# Autodesk Inventor assembly: Ariadna_&_Konarm
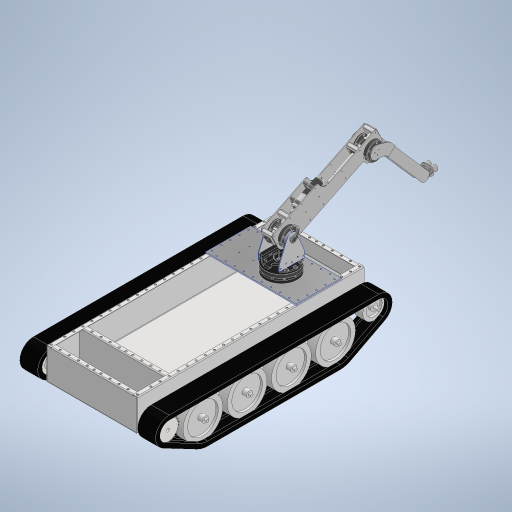
[picture p0: Inventor's stored thumbnail of the model, 512x512]
Saved by Autodesk Inventor 2023 (Build 270158000, 158)
## iProperties
Created: 2023-02-13
Part Number: Ariadna_&_Konarm
Document SubType Name: Assembly
Designer: Kamil
Author: Kamil
## Documents named in this file (3)
- C:\Users\Kamil\Desktop\KONARM\Ariadna_&_Konarm.iam
- C:\Users\Kamil\Desktop\KONARM\Sonsna light\Assembly1.iam
- C:\Users\Kamil\Desktop\KONARM\KONARM_CALY.iam
## Components (2 placed, 2 different names)
1. Assembly1:1 [sub-assembly] — Równoległe:1, Zestawiające:1, Równoległe:2
2. KONARM_CALY:1 [sub-assembly] — Równoległe:1, Zestawiające:1, Równoległe:2
## Relationships (3: Flush 2, Mate 1)
- Równoległe:1 [Flush] (100 mm): Assembly1:1 ↔ KONARM_CALY:1
- Zestawiające:1 [Mate]: Assembly1:1 ↔ KONARM_CALY:1
- Równoległe:2 [Flush]: Assembly1:1 ↔ KONARM_CALY:1
